# Autodesk Inventor assembly: Assembly6
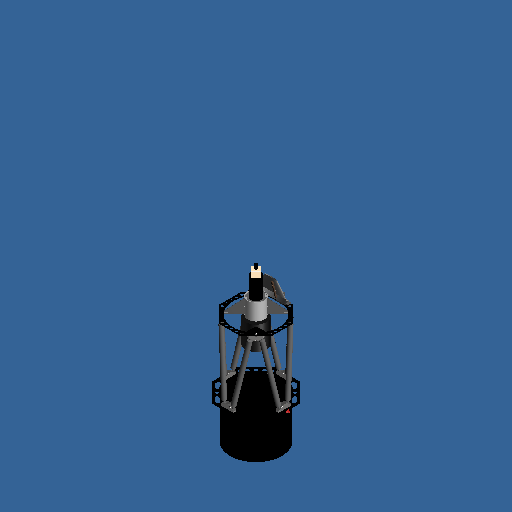
[picture p0: Inventor's stored thumbnail of the model, 512x512]
Saved by Autodesk Inventor 2026.2 (Build 302298000, 298)
## iProperties
Created: 2025-12-09
Part Number: Assembly6
Document SubType Name: Assembly
Designer: Thoma
Mass: 27295.5 g
Surface Area: 25498 cm^2
Volume: 10830.6 cm^3
Density: 2.52023 g/cm^3
Author: Thoma
## Documents named in this file (31)
- C:\Users\Thoma\OneDrive\Desktop\dir\telescope_cover\main\version_2\Main_v3.5.iam
- C:\Users\Thoma\OneDrive\Desktop\dir\telescope_cover\telescope\version_3\Telescope_End.ipt
- C:\Users\Thoma\OneDrive\Desktop\dir\telescope_cover\telescope\version_3\Triangle.ipt
- C:\Users\Thoma\OneDrive\Desktop\dir\telescope_cover\telescope\version_3\Triangle_Bracket_Top.ipt
- C:\Users\Thoma\OneDrive\Desktop\dir\telescope_cover\telescope\version_3\Carbon_Fibre.ipt
- C:\Users\Thoma\OneDrive\Desktop\dir\telescope_cover\telescope\version_3\5mm Screw.ipt
- C:\Users\Thoma\OneDrive\Desktop\dir\telescope_cover\telescope\version_3\35mm_bolt.ipt
- C:\Users\Thoma\OneDrive\Desktop\dir\telescope_cover\telescope\version_3\Triangle_Bracket_Bottom_MIR.ipt
- C:\Users\Thoma\OneDrive\Desktop\dir\telescope_cover\telescope\version_3\Telescope_Base.ipt
- C:\Users\Thoma\OneDrive\Desktop\dir\telescope_cover\telescope\version_3\Full_shaft_Simplify_3.ipt
- C:\Users\Thoma\OneDrive\Desktop\dir\telescope_cover\cover\Conic_Cover_Simplify_1.ipt
- C:\Users\Thoma\OneDrive\Desktop\dir\telescope_cover\telescope\version_3\30mm_bolt.ipt
- C:\Users\Thoma\OneDrive\Desktop\dir\telescope_cover\telescope\version_3\Baffle.ipt
- C:\Users\Thoma\OneDrive\Desktop\dir\telescope_cover\telescope\version_3\Bottom_End_Top.ipt
- C:\Users\Thoma\OneDrive\Desktop\dir\telescope_cover\telescope\version_3\Laser.ipt
- C:\Users\Thoma\OneDrive\Desktop\dir\telescope_cover\cover\rod_v10.ipt
- C:\Users\Thoma\OneDrive\Desktop\dir\telescope_cover\servo\DSS-M15S Servo.ipt
- C:\Users\Thoma\OneDrive\Desktop\dir\telescope_cover\cover\Base_Plate_bottom.ipt
- C:\Users\Thoma\OneDrive\Desktop\dir\telescope_cover\cover\pawn.ipt
- C:\Users\Thoma\OneDrive\Desktop\dir\telescope_cover\screws\m4 threaded insert\m4 threaded insert\m4 threaded insert.ipt
- C:\Users\Thoma\OneDrive\Desktop\dir\telescope_cover\screws\M4 Washer - 9.0 x 0.9 - Black\M4 Washer - 9.0 x 0.9 - Black\M4 Washer - 9.0 x 0.9 - Black.ipt
- C:\Users\Thoma\OneDrive\Desktop\dir\telescope_cover\screws\Screw_DIN_912_M4x12F_A2\Screw_DIN_912_M4x12F_A2\Screw_DIN_912_M4x12F_A2.ipt
- C:\Users\Thoma\OneDrive\Desktop\dir\telescope_cover\cover\Cover_Lower_v4.ipt
- C:\Users\Thoma\OneDrive\Desktop\dir\telescope_cover\screws\M2_Insert.ipt
- C:\Users\Thoma\OneDrive\Desktop\dir\telescope_cover\screws\washer_bossard_m2-5_1170171.ipt
- C:\Users\Thoma\OneDrive\Desktop\dir\telescope_cover\screws\Screw_DIN_912_M2x5F_A2.ipt
- C:\Users\Thoma\OneDrive\Desktop\dir\telescope_cover\screws\Screw_DIN_912_M3x8F_A2\Screw_DIN_912_M3x8F_A2\Screw_DIN_912_M3x8F_A2.ipt
- C:\Users\Thoma\OneDrive\Desktop\dir\telescope_cover\cover\base_plate_v9.ipt
- C:\Users\Thoma\OneDrive\Desktop\dir\telescope_cover\screws\Screw_DIN_912_M4x16F_A2\Screw_DIN_912_M4x16F_A2\Screw_DIN_912_M4x16F_A2.ipt
- C:\Users\Thoma\OneDrive\Desktop\dir\telescope_cover\screws\nut_m4\nut_m4\nut_m4.ipt
- C:\Users\Thoma\OneDrive\Desktop\dir\telescope_cover\screws\Screw_DIN_912_M4x25_A2\Screw_DIN_912_M4x25_A2\Screw_DIN_912_M4x25_A2.ipt
## Components (91 placed, 30 different names)
1. m4 threaded insert:1 — Mate:455, Flush:453
2. m4 threaded insert:2 — Mate:456, Flush:455
3. m4 threaded insert:3 — Mate:457, Flush:454, Mate:463
4. M4 Washer - 9.0 x 0.9 - Black:1 — Mate:458, Mate:463, Mate:464, Tangent:34
5. M4 Washer - 9.0 x 0.9 - Black:2 — Mate:459, Mate:462
6. M4 Washer - 9.0 x 0.9 - Black:3 — Mate:460, Mate:461, Mate:465
7. Cover_Lower_v4:1 — Mate:464, Mate:465, Tangent:34, Mate:466, Mate:467, Mate:468, Mate:469, Mate:470, Mate:471
8. Screw_DIN_912_M4x12F_A2:1 — Mate:466, Mate:469, Angle:142
9. Screw_DIN_912_M4x12F_A2:2 — Mate:467, Mate:470, Angle:141
10. Screw_DIN_912_M4x12F_A2:3 — Mate:468, Mate:471, Angle:140
11. Base_Plate_bottom:1 — Mate:478, Mate:533, Mate:535, Mate:538, Mate:539, Angle:152, Angle:153, Mate:543, Angle:156
12. M2_Insert:4 — Mate:495, Mate:499
13. M2_Insert:5 — Mate:500
14. M2_Insert:6 — Mate:497, Mate:502
15. M2_Insert:7 — Mate:498, Mate:501
16. washer_bossard_m2-5_1170171:3 — Mate:506
17. washer_bossard_m2-5_1170171:4 — Mate:495, Mate:505
18. washer_bossard_m2-5_1170171:5 — Mate:498, Mate:504
19. washer_bossard_m2-5_1170171:6 — Mate:497, Mate:503
20. Screw_DIN_912_M2x5F_A2:3 — Mate:502, Mate:503
21. Screw_DIN_912_M2x5F_A2:4 — Mate:501, Mate:504
22. Screw_DIN_912_M2x5F_A2:5 — Mate:500, Mate:506
23. Screw_DIN_912_M2x5F_A2:6 — Mate:499, Mate:505
24. Screw_DIN_912_M3x8F_A2:1 — Mate:507, Mate:508, Mate:516, Angle:147
25. base_plate_v9:1 — Mate:509, Mate:510, Mate:511, Mate:512, Mate:513, Mate:514, Angle:147, Mate:517, Mate:522, Mate:531, Mate:532, Mate:536, Mate:537, Mate:541, Mate:542, Angle:154, Angle:155
26. M2_Insert:8 — Flush:457, Mate:519
27. M2_Insert:9 — Flush:458, Mate:520
28. M2_Insert:10 — Flush:459, Mate:521
29. M2_Insert:11 — Flush:456, Mate:518, Mate:522
30. Screw_DIN_912_M4x16F_A2:1 — Mate:531, Mate:532, Mate:534, Mate:535, Angle:155
31. nut_m4:1 — Mate:533, Mate:534, Angle:153
32. Screw_DIN_912_M4x25_A2:1 — Mate:536, Mate:537, Mate:538, Mate:540
33. nut_m4:2 — Mate:543, Mate:544, Angle:156
34. nut_m4:3 — Mate:539, Mate:540, Angle:152
35. Screw_DIN_912_M4x16F_A2:2 — Mate:541, Mate:542, Angle:154, Mate:544
36. Laser:2 — Mate:214, Flush:220, Flush:221
37. Laser:1 — Mate:215, Flush:218, Flush:219
38. Baffle:1 — Mate:83
39. Carbon_Fibre:1 — Mate:7, Mate:11, Flush:1, Mate:12, Mate:13, Mate:14, Mate:15, Mate:62, Flush:2, Flush:3, Flush:4, Flush:5, Mate:83, Mate:92, Mate:93, Mate:96, Mate:97, Mate:98, Mate:100, Mate:123, Mate:124, Mate:125, Mate:213
40. Telescope_Base:1 — Mate:62, Angle:31, Mate:89, Mate:90, Angle:40, Mate:108, Mate:109, Angle:48, Mate:110, Mate:111, Angle:49, Mate:112, Mate:113, Angle:50, Mate:214, Mate:215, Flush:218, Flush:221
41. Telescope_End:1 — Mate:1, Mate:2, Angle:2, Mate:7, Mate:54, Mate:55, Angle:26, Angle:31, Mate:86, Mate:88, Mate:91, Angle:41, Mate:101, Angle:45, Angle:46, Mate:114, Mate:115, Angle:51, Mate:116, Mate:117, Angle:52, Mate:118, Mate:119, Angle:53, Mate:478, Mate:509, Mate:510, Mate:511
42. 30mm_bolt:9 — Mate:217, Mate:218, Angle:83
43. 30mm_bolt:10 — Mate:216, Mate:219, Angle:82
44. Triangle_Bracket_Top:5 — Mate:116, Mate:117, Angle:52, Mate:129, Flush:110, Angle:60
45. Triangle_Bracket_Top:4 — Mate:101, Angle:45, Angle:46, Mate:104, Mate:105, Mate:106, Flush:103, Angle:47
46. Triangle_Bracket_Top:3 — Mate:86, Mate:88, Mate:94, Angle:54, Angle:55, Mate:122, Flush:106, Angle:56
47. Triangle_Bracket_Top:1 — Mate:1, Mate:2, Angle:2, Mate:8, Mate:9, Angle:4, Mate:47, Angle:22, Mate:58
48. Triangle:1 — Mate:8, Mate:9, Angle:4, Mate:11, Flush:1, Angle:5, Angle:6, Mate:46, Mate:70, Mate:71
49. Triangle:5 — Mate:92, Mate:93, Mate:94, Mate:102, Mate:128, Flush:109, Angle:59, Mate:132, Flush:181, Angle:81
50. Triangle:6 — Mate:96, Mate:97, Mate:98, Flush:102, Angle:44, Mate:103, Mate:104, Mate:105, Mate:107
51. Triangle:7 — Mate:123, Mate:124, Mate:125, Mate:126, Flush:107, Angle:57, Mate:127, Flush:108, Angle:58, Mate:130, Mate:131
52. 35mm_bolt:6 — Mate:122, Flush:106, Angle:56
53. 35mm_bolt:7 — Mate:129, Flush:110, Angle:60
54. 35mm_bolt:4 — Mate:46, Mate:47, Angle:22
55. 35mm_bolt:5 — Mate:106, Flush:103, Angle:47
56. 5mm Screw:9 — Mate:100, Flush:102, Angle:44
57. 5mm Screw:13 — Mate:213, Flush:181, Angle:81
58. 5mm Screw:10 — Mate:126, Flush:107, Angle:57
59. 5mm Screw:2 — Mate:14, Mate:15, Angle:6
60. 5mm Screw:1 — Mate:12, Mate:13, Angle:5
61. 5mm Screw:11 — Mate:127, Flush:108, Angle:58
62. 5mm Screw:12 — Mate:128, Flush:109, Angle:59
63. Full_shaft_Simplify_3:1
64. Full_shaft_Simplify_3:2 — Tangent:26
65. Full_shaft_Simplify_3:3
66. Full_shaft_Simplify_3:4
67. Full_shaft_Simplify_3:5
68. Full_shaft_Simplify_3:6
69. Full_shaft_Simplify_3:7
70. Full_shaft_Simplify_3:8 — Tangent:31, Tangent:33
71. 30mm_bolt:7 — Mate:120, Flush:104, Angle:54
72. 30mm_bolt:1 — Mate:121, Flush:105, Angle:55
73. 30mm_bolt:8 — Mate:80, Flush:13, Angle:39
74. 30mm_bolt:6 — Mate:78, Flush:11, Angle:37
75. 30mm_bolt:3 — Mate:79, Flush:12, Angle:38
76. 30mm_bolt:2 — Mate:77, Flush:10, Angle:36
77. Triangle_Bracket_Bottom_MIR:4 — Mate:118, Mate:119, Angle:53, Mate:216, Mate:217, Mate:218, Mate:219, Angle:82, Angle:83
78. Triangle_Bracket_Bottom_MIR:3 — Mate:114, Mate:115, Angle:51, Mate:120, Flush:104, Mate:121, Flush:105
79. Triangle_Bracket_Bottom_MIR:2 — Mate:55, Mate:58, Angle:26, Mate:77, Flush:10, Angle:36, Mate:78, Flush:11, Angle:37, Tangent:31
80. Triangle_Bracket_Bottom_MIR:1 — Mate:54, Mate:79, Flush:12, Angle:38, Mate:80, Flush:13, Angle:39, Mate:91, Angle:41
81. Bottom_End_Top:4 — Mate:112, Mate:113, Angle:50, Tangent:26, Tangent:33
82. Bottom_End_Top:3 — Mate:110, Mate:111, Angle:49, Flush:219
83. Bottom_End_Top:2 — Mate:108, Mate:109, Angle:48
84. Bottom_End_Top:1 — Mate:89, Mate:90, Angle:40, Flush:220
85. Conic_Cover_Simplify_1:1 — Flush:2, Mate:131, Mate:132
86. Conic_Cover_Simplify_1:2 — Flush:3, Mate:102, Mate:103
87. Conic_Cover_Simplify_1:3 — Flush:4, Mate:70, Mate:107
88. Conic_Cover_Simplify_1:4 — Mate:71, Flush:5, Mate:130
89. pawn:1 — Mate:419, Mate:517, Flush:456, Mate:518, Flush:457, Mate:519, Flush:458, Mate:520, Flush:459, Mate:521
90. DSS-M15S Servo:1 — Mate:512, Mate:513, Mate:514, Mate:515, Mate:516
91. rod_v10:2 — Mate:419, Mate:455, Flush:453, Mate:456, Mate:457, Flush:454, Flush:455, Mate:458, Mate:459, Mate:460, Mate:461, Mate:462, Angle:140, Angle:141, Angle:142, Mate:507, Mate:508, Mate:515
## Relationships (210: Mate 134, Angle 42, Flush 30, Tangent 4)
- Mate:1: Telescope_End:1 ↔ Triangle_Bracket_Top:1
- Mate:2: Telescope_End:1 ↔ Triangle_Bracket_Top:1
- Angle:2 (0 deg): Telescope_End:1 ↔ Triangle_Bracket_Top:1
- Mate:7: Carbon_Fibre:1 ↔ Telescope_End:1
- Mate:8: Triangle_Bracket_Top:1 ↔ Triangle:1
- Mate:9: Triangle_Bracket_Top:1 ↔ Triangle:1
- Angle:4 (0 deg): Triangle_Bracket_Top:1 ↔ Triangle:1
- Mate:11: Carbon_Fibre:1 ↔ Triangle:1
- Flush:1: Carbon_Fibre:1 ↔ Triangle:1
- Mate:12: Carbon_Fibre:1 ↔ 5mm Screw:1
- Mate:13: Carbon_Fibre:1 ↔ 5mm Screw:1
- Angle:5 (0 deg): Triangle:1 ↔ 5mm Screw:1
- Mate:14: Carbon_Fibre:1 ↔ 5mm Screw:2
- Mate:15: Carbon_Fibre:1 ↔ 5mm Screw:2
- Angle:6 (0 deg): Triangle:1 ↔ 5mm Screw:2
- Mate:46: Triangle:1 ↔ 35mm_bolt:4
- Mate:47: Triangle_Bracket_Top:1 ↔ 35mm_bolt:4
- Angle:22 (0 deg): Triangle_Bracket_Top:1 ↔ 35mm_bolt:4
- Mate:54: Telescope_End:1 ↔ Triangle_Bracket_Bottom_MIR:1
- Mate:55: Telescope_End:1 ↔ Triangle_Bracket_Bottom_MIR:2
- Mate:58: Triangle_Bracket_Top:1 ↔ Triangle_Bracket_Bottom_MIR:2
- Angle:26 (0 deg): Telescope_End:1 ↔ Triangle_Bracket_Bottom_MIR:2
- Mate:62: Carbon_Fibre:1 ↔ Telescope_Base:1
- Angle:31 (0 deg): Telescope_Base:1 ↔ Telescope_End:1
- Flush:2: Carbon_Fibre:1 ↔ Conic_Cover_Simplify_1:1
- Flush:3: Carbon_Fibre:1 ↔ Conic_Cover_Simplify_1:2
- Flush:4: Carbon_Fibre:1 ↔ Conic_Cover_Simplify_1:3
- Mate:70: Triangle:1 ↔ Conic_Cover_Simplify_1:3
- Mate:71: Triangle:1 ↔ Conic_Cover_Simplify_1:4
- Flush:5: Carbon_Fibre:1 ↔ Conic_Cover_Simplify_1:4
- Mate:77: 30mm_bolt:2 ↔ Triangle_Bracket_Bottom_MIR:2
- Flush:10: 30mm_bolt:2 ↔ Triangle_Bracket_Bottom_MIR:2
- Angle:36 (0 deg): 30mm_bolt:2 ↔ Triangle_Bracket_Bottom_MIR:2
- Mate:78: 30mm_bolt:6 ↔ Triangle_Bracket_Bottom_MIR:2
- Flush:11: 30mm_bolt:6 ↔ Triangle_Bracket_Bottom_MIR:2
- Angle:37 (0 deg): 30mm_bolt:6 ↔ Triangle_Bracket_Bottom_MIR:2
- Mate:79: 30mm_bolt:3 ↔ Triangle_Bracket_Bottom_MIR:1
- Flush:12: 30mm_bolt:3 ↔ Triangle_Bracket_Bottom_MIR:1
- Angle:38 (0 deg): 30mm_bolt:3 ↔ Triangle_Bracket_Bottom_MIR:1
- Mate:80: 30mm_bolt:8 ↔ Triangle_Bracket_Bottom_MIR:1
- Flush:13: 30mm_bolt:8 ↔ Triangle_Bracket_Bottom_MIR:1
- Angle:39 (0 deg): 30mm_bolt:8 ↔ Triangle_Bracket_Bottom_MIR:1
- Mate:83: Baffle:1 ↔ Carbon_Fibre:1
- Mate:86: Telescope_End:1 ↔ Triangle_Bracket_Top:3
- Mate:88: Telescope_End:1 ↔ Triangle_Bracket_Top:3
- Mate:89: Telescope_Base:1 ↔ Bottom_End_Top:1
- Mate:90: Telescope_Base:1 ↔ Bottom_End_Top:1
- Angle:40 (0 deg): Telescope_Base:1 ↔ Bottom_End_Top:1
- Mate:91: Telescope_End:1 ↔ Triangle_Bracket_Bottom_MIR:1
- Angle:41 (0 deg): Telescope_End:1 ↔ Triangle_Bracket_Bottom_MIR:1
- Mate:92: Carbon_Fibre:1 ↔ Triangle:5
- Mate:93: Carbon_Fibre:1 ↔ Triangle:5
- Mate:94: Triangle_Bracket_Top:3 ↔ Triangle:5
- Mate:96: Carbon_Fibre:1 ↔ Triangle:6
- Mate:97: Carbon_Fibre:1 ↔ Triangle:6
- Mate:98: Carbon_Fibre:1 ↔ Triangle:6
- Mate:100: Carbon_Fibre:1 ↔ 5mm Screw:9
- Flush:102: Triangle:6 ↔ 5mm Screw:9
- Angle:44 (0 deg): Triangle:6 ↔ 5mm Screw:9
- Mate:101: Telescope_End:1 ↔ Triangle_Bracket_Top:4
- Angle:45 (0 deg): Telescope_End:1 ↔ Triangle_Bracket_Top:4
- Mate:102: Triangle:5 ↔ Conic_Cover_Simplify_1:2
- Mate:103: Triangle:6 ↔ Conic_Cover_Simplify_1:2
- Angle:46 (0 deg): Telescope_End:1 ↔ Triangle_Bracket_Top:4
- Mate:104: Triangle_Bracket_Top:4 ↔ Triangle:6
- Mate:105: Triangle_Bracket_Top:4 ↔ Triangle:6
- Mate:106: Triangle_Bracket_Top:4 ↔ 35mm_bolt:5
- Flush:103: Triangle_Bracket_Top:4 ↔ 35mm_bolt:5
- Angle:47 (0 deg): Triangle_Bracket_Top:4 ↔ 35mm_bolt:5
- Mate:107: Triangle:6 ↔ Conic_Cover_Simplify_1:3
- Mate:108: Telescope_Base:1 ↔ Bottom_End_Top:2
- Mate:109: Telescope_Base:1 ↔ Bottom_End_Top:2
- Angle:48 (0 deg): Telescope_Base:1 ↔ Bottom_End_Top:2
- Mate:110: Telescope_Base:1 ↔ Bottom_End_Top:3
- Mate:111: Telescope_Base:1 ↔ Bottom_End_Top:3
- Angle:49 (0 deg): Telescope_Base:1 ↔ Bottom_End_Top:3
- Mate:112: Telescope_Base:1 ↔ Bottom_End_Top:4
- Mate:113: Telescope_Base:1 ↔ Bottom_End_Top:4
- Angle:50 (0 deg): Telescope_Base:1 ↔ Bottom_End_Top:4
- Mate:114: Telescope_End:1 ↔ Triangle_Bracket_Bottom_MIR:3
- Mate:115: Telescope_End:1 ↔ Triangle_Bracket_Bottom_MIR:3
- Angle:51 (0 deg): Telescope_End:1 ↔ Triangle_Bracket_Bottom_MIR:3
- Mate:116: Telescope_End:1 ↔ Triangle_Bracket_Top:5
- Mate:117: Telescope_End:1 ↔ Triangle_Bracket_Top:5
- Angle:52 (0 deg): Telescope_End:1 ↔ Triangle_Bracket_Top:5
- Mate:118: Telescope_End:1 ↔ Triangle_Bracket_Bottom_MIR:4
- Mate:119: Telescope_End:1 ↔ Triangle_Bracket_Bottom_MIR:4
- Angle:53 (0 deg): Telescope_End:1 ↔ Triangle_Bracket_Bottom_MIR:4
- Mate:120: 30mm_bolt:7 ↔ Triangle_Bracket_Bottom_MIR:3
- Flush:104: 30mm_bolt:7 ↔ Triangle_Bracket_Bottom_MIR:3
- Angle:54 (0 deg): Triangle_Bracket_Top:3 ↔ 30mm_bolt:7
- Mate:121: 30mm_bolt:1 ↔ Triangle_Bracket_Bottom_MIR:3
- Flush:105: 30mm_bolt:1 ↔ Triangle_Bracket_Bottom_MIR:3
- Angle:55 (0 deg): Triangle_Bracket_Top:3 ↔ 30mm_bolt:1
- Mate:122: Triangle_Bracket_Top:3 ↔ 35mm_bolt:6
- Flush:106: Triangle_Bracket_Top:3 ↔ 35mm_bolt:6
- Angle:56 (0 deg): Triangle_Bracket_Top:3 ↔ 35mm_bolt:6
- Mate:123: Carbon_Fibre:1 ↔ Triangle:7
- Mate:124: Carbon_Fibre:1 ↔ Triangle:7
- Mate:125: Carbon_Fibre:1 ↔ Triangle:7
- Mate:126: Triangle:7 ↔ 5mm Screw:10
- Flush:107: Triangle:7 ↔ 5mm Screw:10
- Angle:57 (0 deg): Triangle:7 ↔ 5mm Screw:10
- Mate:127: Triangle:7 ↔ 5mm Screw:11
- Flush:108: Triangle:7 ↔ 5mm Screw:11
- Angle:58 (0 deg): Triangle:7 ↔ 5mm Screw:11
- Mate:128: Triangle:5 ↔ 5mm Screw:12
- Flush:109: Triangle:5 ↔ 5mm Screw:12
- Angle:59 (0 deg): Triangle:5 ↔ 5mm Screw:12
- Mate:129: Triangle_Bracket_Top:5 ↔ 35mm_bolt:7
- Flush:110: Triangle_Bracket_Top:5 ↔ 35mm_bolt:7
- Angle:60 (0 deg): Triangle_Bracket_Top:5 ↔ 35mm_bolt:7
- Mate:130: Triangle:7 ↔ Conic_Cover_Simplify_1:4
- Mate:131: Triangle:7 ↔ Conic_Cover_Simplify_1:1
- Mate:132: Triangle:5 ↔ Conic_Cover_Simplify_1:1
- Mate:213: Carbon_Fibre:1 ↔ 5mm Screw:13
- Flush:181: Triangle:5 ↔ 5mm Screw:13
- Angle:81 (0 deg): Triangle:5 ↔ 5mm Screw:13
- Mate:214: Laser:2 ↔ Telescope_Base:1
- Mate:215: Laser:1 ↔ Telescope_Base:1
- Flush:218: Laser:1 ↔ Telescope_Base:1
- Flush:219 (39.316 mm): Laser:1 ↔ Bottom_End_Top:3
- Flush:220 (39.316 mm): Laser:2 ↔ Bottom_End_Top:1
- Flush:221: Laser:2 ↔ Telescope_Base:1
- Tangent:26: Full_shaft_Simplify_3:2 ↔ Bottom_End_Top:4
- Tangent:31: Full_shaft_Simplify_3:8 ↔ Triangle_Bracket_Bottom_MIR:2
- Tangent:33: Full_shaft_Simplify_3:8 ↔ Bottom_End_Top:4
- Mate:216: 30mm_bolt:10 ↔ Triangle_Bracket_Bottom_MIR:4
- Mate:217: 30mm_bolt:9 ↔ Triangle_Bracket_Bottom_MIR:4
- Mate:218: 30mm_bolt:9 ↔ Triangle_Bracket_Bottom_MIR:4
- Mate:219: 30mm_bolt:10 ↔ Triangle_Bracket_Bottom_MIR:4
- Angle:82 (0 deg): 30mm_bolt:10 ↔ Triangle_Bracket_Bottom_MIR:4
- Angle:83 (0 deg): 30mm_bolt:9 ↔ Triangle_Bracket_Bottom_MIR:4
- Mate:419 (0.5 mm): pawn:1 ↔ rod_v10:2
- Mate:455: m4 threaded insert:1 ↔ rod_v10:2
- Flush:453 (0.2 mm): m4 threaded insert:1 ↔ rod_v10:2
- Mate:456: m4 threaded insert:2 ↔ rod_v10:2
- Mate:457: m4 threaded insert:3 ↔ rod_v10:2
- Flush:454 (0.2 mm): m4 threaded insert:3 ↔ rod_v10:2
- Flush:455 (0.2 mm): m4 threaded insert:2 ↔ rod_v10:2
- Mate:458: M4 Washer - 9.0 x 0.9 - Black:1 ↔ rod_v10:2
- Mate:459: M4 Washer - 9.0 x 0.9 - Black:2 ↔ rod_v10:2
- Mate:460: M4 Washer - 9.0 x 0.9 - Black:3 ↔ rod_v10:2
- Mate:461: M4 Washer - 9.0 x 0.9 - Black:3 ↔ rod_v10:2
- Mate:462: M4 Washer - 9.0 x 0.9 - Black:2 ↔ rod_v10:2
- Mate:463: m4 threaded insert:3 ↔ M4 Washer - 9.0 x 0.9 - Black:1
- Mate:464: M4 Washer - 9.0 x 0.9 - Black:1 ↔ Cover_Lower_v4:1
- Mate:465: M4 Washer - 9.0 x 0.9 - Black:3 ↔ Cover_Lower_v4:1
- Tangent:34: M4 Washer - 9.0 x 0.9 - Black:1 ↔ Cover_Lower_v4:1
- Mate:466: Cover_Lower_v4:1 ↔ Screw_DIN_912_M4x12F_A2:1
- Mate:467: Cover_Lower_v4:1 ↔ Screw_DIN_912_M4x12F_A2:2
- Mate:468: Cover_Lower_v4:1 ↔ Screw_DIN_912_M4x12F_A2:3
- Mate:469: Cover_Lower_v4:1 ↔ Screw_DIN_912_M4x12F_A2:1
- Mate:470: Cover_Lower_v4:1 ↔ Screw_DIN_912_M4x12F_A2:2
- Mate:471: Cover_Lower_v4:1 ↔ Screw_DIN_912_M4x12F_A2:3
- Angle:140 (0 deg): Screw_DIN_912_M4x12F_A2:3 ↔ rod_v10:2
- Angle:141 (0 deg): Screw_DIN_912_M4x12F_A2:2 ↔ rod_v10:2
- Angle:142 (0 deg): Screw_DIN_912_M4x12F_A2:1 ↔ rod_v10:2
- Mate:478: Base_Plate_bottom:1 ↔ Telescope_End:1
- Mate:495: M2_Insert:4 ↔ washer_bossard_m2-5_1170171:4
- Mate:497: M2_Insert:6 ↔ washer_bossard_m2-5_1170171:6
- Mate:498: M2_Insert:7 ↔ washer_bossard_m2-5_1170171:5
- Mate:499: M2_Insert:4 ↔ Screw_DIN_912_M2x5F_A2:6
- Mate:500: M2_Insert:5 ↔ Screw_DIN_912_M2x5F_A2:5
- Mate:501: M2_Insert:7 ↔ Screw_DIN_912_M2x5F_A2:4
- Mate:502: M2_Insert:6 ↔ Screw_DIN_912_M2x5F_A2:3
- Mate:503: washer_bossard_m2-5_1170171:6 ↔ Screw_DIN_912_M2x5F_A2:3
- Mate:504: washer_bossard_m2-5_1170171:5 ↔ Screw_DIN_912_M2x5F_A2:4
- Mate:505: washer_bossard_m2-5_1170171:4 ↔ Screw_DIN_912_M2x5F_A2:6
- Mate:506: washer_bossard_m2-5_1170171:3 ↔ Screw_DIN_912_M2x5F_A2:5
- Mate:507: Screw_DIN_912_M3x8F_A2:1 ↔ rod_v10:2
- Mate:508: Screw_DIN_912_M3x8F_A2:1 ↔ rod_v10:2
- Mate:509: base_plate_v9:1 ↔ Telescope_End:1
- Mate:510: base_plate_v9:1 ↔ Telescope_End:1
- Mate:511: base_plate_v9:1 ↔ Telescope_End:1
- Mate:512: base_plate_v9:1 ↔ DSS-M15S Servo:1
- Mate:513 (1.1 mm): base_plate_v9:1 ↔ DSS-M15S Servo:1
- Mate:514: base_plate_v9:1 ↔ DSS-M15S Servo:1
- Mate:515: DSS-M15S Servo:1 ↔ rod_v10:2
- Mate:516: Screw_DIN_912_M3x8F_A2:1 ↔ DSS-M15S Servo:1
- Angle:147 (0 deg): Screw_DIN_912_M3x8F_A2:1 ↔ base_plate_v9:1
- Mate:517: base_plate_v9:1 ↔ pawn:1
- Flush:456 (0.05 mm): M2_Insert:11 ↔ pawn:1
- Mate:518: M2_Insert:11 ↔ pawn:1
- Flush:457 (0.05 mm): M2_Insert:8 ↔ pawn:1
- Mate:519: M2_Insert:8 ↔ pawn:1
- Flush:458 (0.05 mm): M2_Insert:9 ↔ pawn:1
- Mate:520: M2_Insert:9 ↔ pawn:1
- Flush:459 (0.05 mm): M2_Insert:10 ↔ pawn:1
- Mate:521: M2_Insert:10 ↔ pawn:1
- Mate:522: base_plate_v9:1 ↔ M2_Insert:11
- Mate:531: base_plate_v9:1 ↔ Screw_DIN_912_M4x16F_A2:1
- Mate:532: base_plate_v9:1 ↔ Screw_DIN_912_M4x16F_A2:1
- Mate:533: Base_Plate_bottom:1 ↔ nut_m4:1
- Mate:534: Screw_DIN_912_M4x16F_A2:1 ↔ nut_m4:1
- Mate:535: Base_Plate_bottom:1 ↔ Screw_DIN_912_M4x16F_A2:1
- Mate:536: base_plate_v9:1 ↔ Screw_DIN_912_M4x25_A2:1
- Mate:537: base_plate_v9:1 ↔ Screw_DIN_912_M4x25_A2:1
- Mate:538: Base_Plate_bottom:1 ↔ Screw_DIN_912_M4x25_A2:1
- Mate:539: Base_Plate_bottom:1 ↔ nut_m4:3
- Mate:540: Screw_DIN_912_M4x25_A2:1 ↔ nut_m4:3
- Angle:152 (0 deg): Base_Plate_bottom:1 ↔ nut_m4:3
- Angle:153 (0 deg): Base_Plate_bottom:1 ↔ nut_m4:1
- Mate:541: base_plate_v9:1 ↔ Screw_DIN_912_M4x16F_A2:2
- Mate:542: base_plate_v9:1 ↔ Screw_DIN_912_M4x16F_A2:2
- Angle:154 (0 deg): base_plate_v9:1 ↔ Screw_DIN_912_M4x16F_A2:2
- Angle:155 (0 deg): base_plate_v9:1 ↔ Screw_DIN_912_M4x16F_A2:1
- Mate:543: Base_Plate_bottom:1 ↔ nut_m4:2
- Mate:544: nut_m4:2 ↔ Screw_DIN_912_M4x16F_A2:2
- Angle:156 (0 deg): Base_Plate_bottom:1 ↔ nut_m4:2
